# Autodesk Inventor assembly: Mecanum Wheel
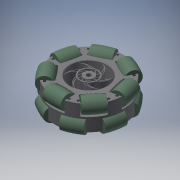
[picture p0: Inventor's stored thumbnail of the model, 180x180]
Saved by Autodesk Inventor 2018 (Build 220112000, 112)
## iProperties
Created: 2018-03-28
Part Number: Mecanum Wheel
Document SubType Name: Assembly
Designer: Ajith Thomas
Author: Ajith Thomas
## Documents named in this file (3)
- C:\Users\Ajith Thomas\Dropbox\Gas_Sensing_Robot\FumeBot-Design\Mecanum\Mecanum Wheel.iam
- C:\Users\Ajith Thomas\Dropbox\Gas_Sensing_Robot\FumeBot-Design\Mecanum\Mecanum Hub.ipt
- C:\Users\Ajith Thomas\Dropbox\Gas_Sensing_Robot\FumeBot-Design\Mecanum\Mechnum small wheel.ipt
## Components (15 placed, 2 different names)
1. Mecanum Hub:1 — Mate:1, Tangent:1, Tangent:2, Mate:2, Tangent:3, Tangent:4, Mate:3, Tangent:5, Tangent:6, Mate:4, Tangent:7, Tangent:8, Mate:5, Tangent:9, Tangent:10, Mate:6, Tangent:11, Tangent:12, Mate:7, Tangent:13, Tangent:14, Mate:8, Tangent:15, Tangent:16, Mate:9, Tangent:17, Tangent:18, Mate:10, Tangent:19, Tangent:20, Mate:11, Tangent:21, Tangent:22, Mate:12, Tangent:23, Tangent:24, Mate:13, Tangent:25, Tangent:26, Mate:14, Tangent:27, Tangent:28
2. Mechnum small wheel:1 — Mate:1, Tangent:1, Tangent:2
3. Mechnum small wheel:2 — Mate:5, Tangent:9, Tangent:10
4. Mechnum small wheel:3 — Mate:2, Tangent:3, Tangent:4
5. Mechnum small wheel:4 — Mate:6, Tangent:11, Tangent:12
6. Mechnum small wheel:5 — Mate:3, Tangent:5, Tangent:6
7. Mechnum small wheel:6 — Mate:7, Tangent:13, Tangent:14
8. Mechnum small wheel:7 — Mate:4, Tangent:7, Tangent:8
9. Mechnum small wheel:8 — Mate:12, Tangent:23, Tangent:24
10. Mechnum small wheel:9 — Mate:13, Tangent:25, Tangent:26
11. Mechnum small wheel:10 — Mate:14, Tangent:27, Tangent:28
12. Mechnum small wheel:11 — Mate:11, Tangent:21, Tangent:22
13. Mechnum small wheel:12 — Mate:10, Tangent:19, Tangent:20
14. Mechnum small wheel:13 — Mate:8, Tangent:15, Tangent:16
15. Mechnum small wheel:14 — Mate:9, Tangent:17, Tangent:18
## Relationships (42: Tangent 28, Mate 14)
- Mate:1: Mecanum Hub:1 ↔ Mechnum small wheel:1
- Tangent:1: Mecanum Hub:1 ↔ Mechnum small wheel:1
- Tangent:2: Mecanum Hub:1 ↔ Mechnum small wheel:1
- Mate:2: Mecanum Hub:1 ↔ Mechnum small wheel:3
- Tangent:3: Mecanum Hub:1 ↔ Mechnum small wheel:3
- Tangent:4: Mecanum Hub:1 ↔ Mechnum small wheel:3
- Mate:3: Mecanum Hub:1 ↔ Mechnum small wheel:5
- Tangent:5: Mecanum Hub:1 ↔ Mechnum small wheel:5
- Tangent:6: Mecanum Hub:1 ↔ Mechnum small wheel:5
- Mate:4: Mecanum Hub:1 ↔ Mechnum small wheel:7
- Tangent:7: Mecanum Hub:1 ↔ Mechnum small wheel:7
- Tangent:8: Mecanum Hub:1 ↔ Mechnum small wheel:7
- Mate:5: Mecanum Hub:1 ↔ Mechnum small wheel:2
- Tangent:9: Mecanum Hub:1 ↔ Mechnum small wheel:2
- Tangent:10: Mecanum Hub:1 ↔ Mechnum small wheel:2
- Mate:6: Mecanum Hub:1 ↔ Mechnum small wheel:4
- Tangent:11: Mecanum Hub:1 ↔ Mechnum small wheel:4
- Tangent:12: Mecanum Hub:1 ↔ Mechnum small wheel:4
- Mate:7: Mecanum Hub:1 ↔ Mechnum small wheel:6
- Tangent:13: Mecanum Hub:1 ↔ Mechnum small wheel:6
- Tangent:14: Mecanum Hub:1 ↔ Mechnum small wheel:6
- Mate:8: Mecanum Hub:1 ↔ Mechnum small wheel:13
- Tangent:15: Mecanum Hub:1 ↔ Mechnum small wheel:13
- Tangent:16: Mecanum Hub:1 ↔ Mechnum small wheel:13
- Mate:9: Mecanum Hub:1 ↔ Mechnum small wheel:14
- Tangent:17: Mecanum Hub:1 ↔ Mechnum small wheel:14
- Tangent:18: Mecanum Hub:1 ↔ Mechnum small wheel:14
- Mate:10: Mecanum Hub:1 ↔ Mechnum small wheel:12
- Tangent:19: Mecanum Hub:1 ↔ Mechnum small wheel:12
- Tangent:20: Mecanum Hub:1 ↔ Mechnum small wheel:12
- Mate:11: Mecanum Hub:1 ↔ Mechnum small wheel:11
- Tangent:21: Mecanum Hub:1 ↔ Mechnum small wheel:11
- Tangent:22: Mecanum Hub:1 ↔ Mechnum small wheel:11
- Mate:12: Mecanum Hub:1 ↔ Mechnum small wheel:8
- Tangent:23: Mecanum Hub:1 ↔ Mechnum small wheel:8
- Tangent:24: Mecanum Hub:1 ↔ Mechnum small wheel:8
- Mate:13: Mecanum Hub:1 ↔ Mechnum small wheel:9
- Tangent:25: Mecanum Hub:1 ↔ Mechnum small wheel:9
- Tangent:26: Mecanum Hub:1 ↔ Mechnum small wheel:9
- Mate:14: Mecanum Hub:1 ↔ Mechnum small wheel:10
- Tangent:27: Mecanum Hub:1 ↔ Mechnum small wheel:10
- Tangent:28: Mecanum Hub:1 ↔ Mechnum small wheel:10
